(part 1 of 2)
# Autodesk Inventor assembly: Drive Roller Assembly 2
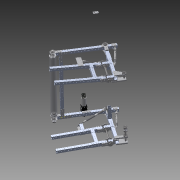
[picture p0: Inventor's stored thumbnail of the model, 180x180]
Saved by Autodesk Inventor 2014 (Build 180170000, 170)
## iProperties
Created: 2014-01-12
Part Number: Drive Roller Assembly 2
Document SubType Name: Assembly
Designer: Michael
Mass: 6489.5 g
Surface Area: 18387.5 cm^2
Volume: 1765.28 cm^3
Density: 3.67619 g/cm^3
Author: Michael
## Documents named in this file (45)
- C:\Users\Michael\Documents\GitHub\2014buildCAD\New Collector\Drive Roller Assembly 2.iam
- C:\Users\Michael\Documents\GitHub\2014buildCAD\Collector\Hex Shaft Collar 1-2 in (7552K500).ipt
- C:\Users\Michael\Documents\GitHub\2014buildCAD\Collector\Roller End Cap Drive (3-D Printed).ipt
- C:\Users\Michael\Documents\GitHub\2014buildCAD\Collector\VersaPlanetary (Fixed).iam
- C:\Users\Michael\Documents\GitHub\2014buildCAD\New Collector\Polycarbonate Roller 2 OD 1-16 Thick (8585K64).ipt
- C:\Users\Michael\Documents\GitHub\2014buildCAD\New Collector\Hex Bearing 1-2 in (FR8ZZ-Hex, am-0279).ipt
- C:\Users\Michael\Documents\GitHub\2014buildCAD\New Collector\Hex Shaft Collar 1-2 in (7552K500).ipt
- C:\Users\Michael\Documents\GitHub\2014buildCAD\New Collector\Roller End Cap Drive (3-D Printed).ipt
- C:\Users\Michael\Documents\GitHub\2014buildCAD\New Collector\Vex Pro End Bearing Mount.ipt
- C:\Users\Michael\Documents\GitHub\2014buildCAD\New Collector\Vex Pro 1x1 rectangular tubing 14 in length.ipt
- C:\Users\Michael\Documents\GitHub\2014buildCAD\New Collector\Hex Shaft Aluminum 1-2 in (am-2291).ipt
- C:\Users\Michael\Documents\GitHub\2014buildCAD\New Collector\Timing Pulley (HTD 5mm) - 18T 9mm Double Flange, 1-2 in Hex (VexPro).ipt
- C:\Users\Michael\Documents\GitHub\2014buildCAD\New Collector\Clamp with Piston Assembly.iam
- C:\Users\Michael\Documents\GitHub\2014buildCAD\New Collector\Vex Pro 90 degree gusset.ipt
- C:\Users\Michael\Documents\GitHub\2014buildCAD\New Collector\Vex Pro 1x1 rectangular tubing 2 in length.ipt
- C:\Users\Michael\Documents\GitHub\2014buildCAD\New Collector\Hex Shaft 3-8 in (am-0855).ipt
- C:\Users\Michael\Documents\GitHub\2014buildCAD\New Collector\Hex Shaft Collar 3-8 in (7552K300).ipt
- C:\Users\Michael\Documents\GitHub\2014buildCAD\New Collector\Hex Shaft 1-2 in (am-0856).ipt
- C:\Users\Michael\Documents\GitHub\2014buildCAD\New Collector\Spacer 2.ipt
- C:\Users\Michael\Documents\GitHub\2014buildCAD\New Collector\Gusset 3 (R-R) (Custom) ipt.ipt
- C:\Users\Michael\Documents\GitHub\2014buildCAD\New Collector\Gusset 3 (L-R) (Custom).ipt
- C:\Users\Michael\Documents\GitHub\2014buildCAD\New Collector\Gusset 3 (L-L) (Custom) ipt.ipt
- C:\Users\Michael\Documents\GitHub\2014buildCAD\New Collector\Gusset 3 (R-L) (Custom).ipt
- C:\Users\Michael\Documents\GitHub\2014buildCAD\New Collector\Vex Pro 1x1 rectangular tubing 4 in length.ipt
- C:\Users\Michael\Documents\GitHub\2014buildCAD\New Collector\Pneumatic Piston Front Flange (Lt Custom).ipt
- C:\Users\Michael\Documents\GitHub\2014buildCAD\New Collector\Pneumatic Piston Front Flange (Rt Custom).ipt
- C:\Users\Michael\Documents\GitHub\2014buildCAD\New Collector\Pneumatic Piston Back Flange (Rt Custom).ipt
- C:\Users\Michael\Documents\GitHub\2014buildCAD\New Collector\Bearing Mount Spacer 1-8 in.ipt
- C:\Users\Michael\Documents\GitHub\2014buildCAD\New Collector\Vex Pro 1x1 rectangular tubing 14 in length (roller).ipt
- C:\Users\Michael\Documents\GitHub\2014buildCAD\New Collector\Pneumatic Piston Back Flange (Right Custom).ipt
- C:\Users\Michael\Documents\GitHub\2014buildCAD\New Collector\Hex Shaft 1-2 in 5 in long (am-0856).ipt
- C:\Users\Michael\Documents\GitHub\2014buildCAD\New Collector\Vex Pro End Bearing Mount (Bolt).ipt
- C:\Users\Michael\Documents\GitHub\2014buildCAD\New Collector\Bracket.ipt
- C:\Users\Michael\Documents\GitHub\2014buildCAD\New Collector\Roller Piston 4 (.5 and 1 in Stroke, 9-16 in Bore).iam
- C:\Users\Michael\Documents\GitHub\2014buildCAD\New Collector\Shaft Collar 3-16 in ID (6435K510).ipt
- C:\Users\Michael\Documents\GitHub\2014buildCAD\New Collector\Standoff #8 (91125A459).ipt
- C:\Users\Michael\Documents\GitHub\2014buildCAD\New Collector\Vex Pro 1x1 rectangular tubing 21.375 in length.ipt
- C:\Users\Michael\Documents\GitHub\2014buildCAD\New Collector\Roller Crossbar Gusset (Custom).ipt
- C:\Users\Michael\Documents\GitHub\2014buildCAD\New Collector\Vex Pro 1x1 rectangular tubing 2 in length (Flange Support).ipt
- C:\Users\Michael\Documents\GitHub\2014buildCAD\New Collector\Vex Pro 90 degree gusset (1-8 in).ipt
- C:\Users\Michael\Documents\GitHub\2014buildCAD\New Collector\Timing Pulley (HTD 5mm) - 18T 15mm 1-2 in Hex.ipt
- C:\Users\Michael\Documents\GitHub\2014buildCAD\New Collector\Hex Spacer.ipt
- C:\Users\Michael\Documents\GitHub\2014buildCAD\New Collector\Side Mount Custom.ipt
- C:\Users\Michael\Documents\GitHub\2014buildCAD\New Collector\Clamp Piston ( 1 in stroke twice, 9-16 bore).iam
- C:\Users\Michael\Documents\GitHub\2014buildCAD\New Collector\Hex Spacer 1-2 .ipt
## Components (138 placed, 42 different names)
1. Roller End Cap Drive (3-D Printed):2 — Mate:154, Mate:155, Mate:157, Mate:158, Mate:466, Mate:469
2. VersaPlanetary (Fixed):1 [sub-assembly] — Mate:113, Mate:114, Mate:120, Mate:121, Mate:153, Mate:990, Mate:991, Mate:992
3. Hex Shaft Collar 1-2 in (7552K500):9 — Mate:113, Mate:114
4. Hex Shaft Collar 1-2 in (7552K500):10 — Mate:120, Mate:121
5. Polycarbonate Roller 2 OD 1-16 Thick (8585K64):3 — Mate:157, Mate:158, Mate:159, Mate:160
6. Hex Bearing 1-2 in (FR8ZZ-Hex, am-0279):3 — Mate:128, Mate:129, Mate:134, Mate:466, Mate:797
7. Roller End Cap Drive (3-D Printed):5 — Mate:159, Mate:160, Mate:632, Mate:635
8. Hex Shaft Aluminum 1-2 in (am-2291):1 — Flush:1, Mate:132, Mate:133, Mate:134, Mate:143, Mate:144, Mate:146, Mate:147, Mate:154, Mate:155, Mate:172, Mate:173, Mate:179, Mate:180, Mate:467, Mate:468, Mate:797
9. Vex Pro End Bearing Mount:4 — Mate:130, Mate:131, Mate:621, Mate:798, Mate:799, Mate:873
10. Vex Pro End Bearing Mount:5 — Mate:128, Mate:129, Mate:624, Mate:800, Mate:801, Mate:866, Mate:867, Mate:868, Mate:869, Mate:870, Mate:871, Mate:872
11. Hex Bearing 1-2 in (FR8ZZ-Hex, am-0279):4 — Mate:130, Mate:131, Flush:1, Mate:132, Mate:133, Mate:161
12. Timing Pulley (HTD 5mm) - 18T 9mm Double Flange, 1-2 in Hex (VexPro):3 — Mate:143, Mate:144, Mate:145, Mate:161
13. Hex Shaft Collar 1-2 in (7552K500):13 — Mate:145, Mate:146, Mate:147, Flush:2
14. Hex Shaft Collar 1-2 in (7552K500):14 — Flush:4, Mate:152
15. Timing Pulley (HTD 5mm) - 18T 9mm Double Flange, 1-2 in Hex (VexPro):4 — Mate:150, Flush:3, Mate:151, Flush:4, Mate:152
16. Hex Shaft Collar 1-2 in (7552K500):15 — Flush:2, Mate:150, Flush:3, Mate:151, Mate:153
17. Hex Bearing 1-2 in (FR8ZZ-Hex, am-0279):5 — Mate:178, Mate:758, Mate:759
18. Vex Pro End Bearing Mount:7 — Mate:631, Mate:804, Mate:805
19. Vex Pro End Bearing Mount:8 — Mate:629, Mate:802, Mate:803, Mate:874, Mate:875, Mate:876, Mate:877, Mate:878, Mate:879, Mate:880, Mate:881
20. Hex Bearing 1-2 in (FR8ZZ-Hex, am-0279):6 — Mate:172, Mate:173, Mate:470, Mate:471, Mate:632
21. Hex Shaft Collar 1-2 in (7552K500):16 — Mate:178, Mate:179, Mate:180, Flush:13
22. Clamp with Piston Assembly:1 [sub-assembly] — Mate:226, Mate:227, Flush:6, Mate:230, Mate:233, Mate:673, Mate:689, Mate:690, Mate:918, Mate:921
23. Vex Pro 1x1 rectangular tubing 14 in length:5 — Mate:203, Mate:210, Mate:211, Mate:221, Mate:222, Mate:223, Mate:427, Mate:429, Flush:20, Mate:653, Mate:940, Mate:942, Mate:975, Mate:979, Mate:981, Mate:983, Mate:1022, Mate:1023, Flush:27, Mate:1053, Mate:1054, Mate:1055
24. Vex Pro 1x1 rectangular tubing 14 in length:6 — Mate:258, Mate:259, Mate:260, Mate:263, Mate:320, Mate:321, Mate:418, Mate:419, Mate:420, Flush:20, Mate:658, Mate:935, Mate:936, Mate:938, Mate:973, Mate:974, Mate:976, Mate:977, Mate:978, Mate:1020, Mate:1021, Flush:26, Mate:1056, Mate:1057, Mate:1058
25. Vex Pro 90 degree gusset:8 — Mate:203, Mate:210, Mate:211, Mate:212, Mate:213, Mate:214
26. Vex Pro 1x1 rectangular tubing 2 in length:1 — Mate:212, Mate:213, Mate:214, Flush:25, Mate:941, Mate:961, Mate:962, Mate:964, Mate:965
27. Vex Pro 90 degree gusset:10 — Mate:221, Mate:222, Mate:223, Mate:433, Mate:434, Mate:435
28. Vex Pro 1x1 rectangular tubing 2 in length:2 — Mate:224, Mate:225, Flush:5, Mate:428, Mate:967, Mate:968, Mate:970, Mate:971
29. Hex Shaft 3-8 in (am-0855):1 — Mate:224, Mate:225, Flush:5, Mate:226, Mate:227, Flush:6, Mate:228, Mate:229, Mate:231, Mate:232, Mate:919, Mate:920, Mate:922, Mate:923, Mate:963, Mate:966, Mate:969, Mate:972
30. Hex Shaft Collar 3-8 in (7552K300):1 — Mate:228, Mate:229, Mate:230
31. Hex Shaft Collar 3-8 in (7552K300):2 — Mate:231, Mate:232, Mate:233
32. Clamp with Piston Assembly:2 [sub-assembly] — Mate:666, Mate:668, Mate:669, Mate:916, Mate:924
33. Vex Pro 90 degree gusset:12 — Mate:263, Mate:320, Mate:321, Mate:324, Mate:325
34. Vex Pro 1x1 rectangular tubing 2 in length:3 — Mate:324, Mate:325, Flush:25, Mate:937, Mate:949, Mate:950, Mate:952, Mate:953
35. Vex Pro 90 degree gusset:13 — Mate:258, Mate:259, Mate:260, Mate:425, Mate:426, Mate:492
36. Vex Pro 1x1 rectangular tubing 2 in length:4 — Mate:955, Mate:956, Mate:958, Mate:959
37. Hex Shaft 3-8 in (am-0855):2 — Mate:915, Mate:917, Mate:925, Mate:926, Mate:951, Mate:954, Mate:957, Mate:960
38. Hex Shaft Collar 3-8 in (7552K300):3
39. Hex Shaft Collar 3-8 in (7552K300):4
40. Vex Pro 90 degree gusset:14 — Mate:476, Mate:477, Mate:478, Mate:653
41. Vex Pro 90 degree gusset:15 — Mate:650, Mate:651, Mate:652, Mate:939, Mate:1022, Mate:1023
42. Vex Pro 90 degree gusset:17 — Mate:485, Mate:486, Mate:487
43. Vex Pro 90 degree gusset:18 — Mate:656, Mate:657, Mate:658, Mate:659, Mate:1020, Mate:1021
44. Hex Shaft 1-2 in (am-0856):2 — Mate:402, Mate:403, Mate:405, Mate:406, Mate:447, Mate:448, Flush:12
45. Hex Shaft Collar 1-2 in (7552K500):18 — Mate:402, Mate:403, Mate:450, Flush:12
46. Hex Shaft Collar 1-2 in (7552K500):19 — Mate:405, Mate:406, Mate:449
47. Hex Shaft Collar 1-2 in (7552K500):20 — Mate:706, Mate:707, Mate:726, Mate:945
48. Hex Shaft Collar 1-2 in (7552K500):21 — Mate:446, Mate:704, Mate:705, Flush:22
49. Spacer 2:1 — Mate:418, Mate:419, Mate:420, Mate:438, Mate:439, Mate:451, Mate:452, Mate:453
50. Gusset 3 (R-R) (Custom) ipt:1 — Mate:425, Mate:426, Mate:446, Mate:492
51. Spacer 2:2 — Mate:427, Mate:428, Mate:429, Mate:430, Mate:431, Mate:455, Mate:456, Mate:457
52. Gusset 3 (L-R) (Custom):1 — Mate:430, Mate:431, Mate:447, Mate:448, Mate:450, Mate:461
53. Gusset 3 (L-L) (Custom) ipt:1 — Mate:433, Mate:434, Mate:435, Mate:449
54. Gusset 3 (R-L) (Custom):1 — Mate:438, Mate:439, Mate:465, Mate:708, Mate:709, Mate:726, Mate:1034
55. Spacer 2:3 — Mate:451, Mate:452, Mate:453, Mate:462, Mate:463, Mate:464
56. Spacer 2:4 — Mate:455, Mate:456, Mate:457, Mate:458, Mate:459, Mate:460
57. Spacer 2:5 — Mate:458, Mate:459, Mate:460, Mate:461
58. Spacer 2:6 — Mate:462, Mate:463, Mate:464, Mate:465
59. Hex Shaft Collar 1-2 in (7552K500):22 — Mate:467, Mate:468, Mate:469
60. Hex Shaft Aluminum 1-2 in (am-2291):2 — Mate:470, Mate:471, Flush:13, Mate:633, Mate:634, Mate:758, Mate:759
61. Vex Pro 1x1 rectangular tubing 4 in length:1 — Mate:476, Mate:477, Mate:478, Mate:650, Mate:651, Mate:652, Mate:683, Mate:684, Mate:685
62. Vex Pro 1x1 rectangular tubing 4 in length:2 — Mate:485, Mate:486, Mate:487, Mate:656, Mate:657, Mate:659, Mate:694, Mate:699, Mate:700
63. Bearing Mount Spacer 1-8 in:1 — Mate:748, Mate:749, Mate:750, Mate:973, Mate:976
64. Bearing Mount Spacer 1-8 in:3 — Mate:743, Mate:744, Mate:745, Mate:974, Mate:978
65. Hex Bearing 1-2 in (FR8ZZ-Hex, am-0279):7 — Flush:15, Mate:560, Mate:561, Flush:23, Mate:754, Mate:755, Mate:830
66. Hex Shaft 1-2 in (am-0856):4 — Mate:560, Mate:561, Mate:562, Mate:563, Flush:23, Mate:774, Mate:829, Mate:831, Mate:833, Mate:834, Mate:1040, Mate:1043
67. Hex Bearing 1-2 in (FR8ZZ-Hex, am-0279):8 — Flush:15, Mate:746, Mate:747, Mate:774, Mate:832
68. Vex Pro 1x1 rectangular tubing 14 in length (roller):1 — Mate:562, Mate:563, Mate:621, Mate:624, Flush:21, Mate:790, Mate:791, Mate:793, Mate:798, Mate:799, Mate:800, Mate:801, Mate:862, Mate:863, Mate:864, Mate:887, Mate:903, Mate:904, Mate:909, Mate:910, Mate:912, Mate:988, Mate:989, Mate:1038, Mate:1039, Mate:1041, Mate:1042, Flush:26, Mate:1050
69. Bearing Mount Spacer 1-8 in:5 — Mate:740, Mate:741, Mate:742, Mate:983
70. Bearing Mount Spacer 1-8 in:7 — Mate:735, Mate:736, Mate:737, Mate:975, Mate:980
71. Hex Bearing 1-2 in (FR8ZZ-Hex, am-0279):9 — Flush:19, Mate:752, Mate:753, Mate:854
72. Hex Shaft 1-2 in (am-0856):5 — Flush:19, Mate:775, Mate:836, Mate:843, Mate:852, Mate:853, Mate:1037, Mate:1046, Mate:1049
73. Hex Bearing 1-2 in (FR8ZZ-Hex, am-0279):10 — Mate:738, Mate:739, Mate:775, Mate:835
74. Vex Pro 1x1 rectangular tubing 14 in length (roller):2 — Mate:629, Mate:631, Flush:21, Mate:802, Mate:803, Mate:804, Mate:805, Mate:806, Mate:807, Mate:808, Mate:809, Mate:810, Mate:811, Mate:892, Mate:896, Mate:905, Mate:906, Mate:907, Mate:908, Mate:1036, Mate:1044, Mate:1045, Mate:1047, Mate:1048, Flush:27
75. Hex Shaft Collar 1-2 in (7552K500):23 — Mate:633, Mate:634, Mate:635
76. Pneumatic Piston Front Flange (Rt Custom):2 — Mate:666, Mate:668, Mate:669, Mate:932, Mate:933, Mate:934, Mate:1051
77. Pneumatic Piston Front Flange (Lt Custom):1 — Mate:673, Mate:689, Mate:690, Mate:929, Mate:930, Mate:931, Mate:1052
78. Pneumatic Piston Back Flange (Rt Custom):1 — Mate:683, Mate:684, Mate:685, Mate:1028, Mate:1029, Mate:1030
79. Pneumatic Piston Back Flange (Right Custom):1 — Mate:694, Mate:699, Mate:700, Mate:1024, Mate:1025, Mate:1026
80. Hex Shaft 1-2 in 5 in long (am-0856):1 — Mate:704, Mate:705, Mate:706, Mate:707, Mate:708, Mate:709, Flush:22, Mate:714, Mate:715, Mate:946, Mate:947, Mate:1032, Mate:1033
81. Hex Shaft Collar 1-2 in (7552K500):24 — Mate:714, Mate:715, Mate:948
82. Vex Pro End Bearing Mount (Bolt):1 — Mate:735, Mate:736, Mate:737, Mate:738, Mate:739, Mate:979, Mate:980
83. Vex Pro End Bearing Mount (Bolt):2 — Mate:740, Mate:741, Mate:742, Mate:752, Mate:753, Mate:981
84. Vex Pro End Bearing Mount (Bolt):3 — Mate:743, Mate:744, Mate:745, Mate:746, Mate:747
85. Vex Pro End Bearing Mount (Bolt):4 — Mate:748, Mate:749, Mate:750, Mate:754, Mate:755, Mate:977
86. Bracket:1 — Mate:790, Mate:791, Mate:793, Mate:860, Mate:1059
87. Bracket:2 — Mate:806, Mate:807, Mate:808, Mate:856, Mate:1060
88. Bracket:3 — Mate:809, Mate:810, Mate:811, Mate:858
89. Hex Shaft Collar 1-2 in (7552K500):25 — Mate:829, Mate:830, Mate:831
90. Hex Shaft Collar 1-2 in (7552K500):26 — Mate:832, Mate:833, Mate:834
91. Hex Shaft Collar 1-2 in (7552K500):27 — Mate:835, Mate:836, Mate:843
92. Hex Shaft Collar 1-2 in (7552K500):29 — Mate:852, Mate:853, Mate:854
93. Shaft Collar 3-16 in ID (6435K510):1 — Mate:858, Mate:1062
94. Shaft Collar 3-16 in ID (6435K510):2 — Mate:856, Mate:1061
95. Shaft Collar 3-16 in ID (6435K510):3 — Mate:860, Mate:1063
96. Shaft Collar 3-16 in ID (6435K510):4 — Mate:865, Mate:1064
97. Bracket:4 — Mate:862, Mate:863, Mate:864, Mate:865
98. Standoff #8 (91125A459):1 — Mate:866, Mate:867
99. Standoff #8 (91125A459):2 — Mate:868, Mate:869
100. Standoff #8 (91125A459):3 — Mate:870, Mate:871
101. Standoff #8 (91125A459):4 — Mate:872, Mate:873
102. Standoff #8 (91125A459):5 — Mate:874, Mate:875
103. Standoff #8 (91125A459):6 — Mate:876, Mate:877
104. Standoff #8 (91125A459):7 — Mate:878, Mate:879
105. Standoff #8 (91125A459):8 — Mate:880, Mate:881
106. Vex Pro 1x1 rectangular tubing 21.375 in length:1 — Mate:894, Mate:897, Mate:900, Mate:901, Mate:902, Mate:911
107. Roller Crossbar Gusset (Custom):2 — Mate:887, Mate:900, Mate:901, Mate:902, Mate:903, Mate:904
108. Roller Crossbar Gusset (Custom):3 — Mate:896, Mate:897, Mate:905, Mate:906
109. Roller Crossbar Gusset (Custom):4 — Mate:892, Mate:894, Mate:907, Mate:908
110. Roller Crossbar Gusset (Custom):5 — Mate:909, Mate:910, Mate:911, Mate:912
111. Hex Shaft Collar 3-8 in (7552K300):5 — Mate:915, Mate:916, Mate:917
112. Hex Shaft Collar 3-8 in (7552K300):6 — Mate:918, Mate:919, Mate:920
113. Hex Shaft Collar 3-8 in (7552K300):7 — Mate:921, Mate:922, Mate:923
114. Hex Shaft Collar 3-8 in (7552K300):8 — Mate:924, Mate:925, Mate:926
115. Vex Pro 1x1 rectangular tubing 2 in length (Flange Support):1 — Mate:929, Mate:930, Mate:931
116. Vex Pro 1x1 rectangular tubing 2 in length (Flange Support):2 — Mate:932, Mate:933, Mate:934
117. Vex Pro 90 degree gusset (1-8 in):1 — Mate:935, Mate:936, Mate:937, Mate:938
118. Vex Pro 90 degree gusset (1-8 in):2 — Mate:939, Mate:940, Mate:941, Mate:942
119. Timing Pulley (HTD 5mm) - 18T 15mm 1-2 in Hex:1 — Mate:945, Mate:946, Mate:947, Mate:948
120. Hex Spacer:1 — Mate:949, Mate:950, Mate:951
121. Hex Spacer:2 — Mate:952, Mate:953, Mate:954
122. Hex Spacer:3 — Mate:955, Mate:956, Mate:957
123. Hex Spacer:4 — Mate:958, Mate:959, Mate:960
124. Hex Spacer:5 — Mate:961, Mate:962, Mate:963
125. Hex Spacer:6 — Mate:964, Mate:965, Mate:966
126. Hex Spacer:7 — Mate:967, Mate:968, Mate:969
127. Hex Spacer:8 — Mate:970, Mate:971, Mate:972
128. Side Mount Custom:1 — Mate:988, Mate:989, Mate:990, Mate:991, Mate:992, Mate:1050
129. Clamp Piston ( 1 in stroke twice, 9-16 bore):1 [sub-assembly] — Mate:1024, Mate:1025, Mate:1026, Mate:1051
130. Clamp Piston ( 1 in stroke twice, 9-16 bore):2 [sub-assembly] — Mate:1028, Mate:1029, Mate:1030, Mate:1052
131. Hex Shaft Collar 1-2 in (7552K500):30 — Mate:1032, Mate:1033, Mate:1034
132. Hex Spacer:9 — Mate:1036, Mate:1037
133. Hex Spacer 1-2 :1 — Mate:1038, Mate:1039, Mate:1040
134. Hex Spacer 1-2 :2 — Mate:1041, Mate:1042, Mate:1043
135. Hex Spacer 1-2 :3 — Mate:1044, Mate:1045, Mate:1046
136. Hex Spacer 1-2 :4 — Mate:1047, Mate:1048, Mate:1049
137. Roller Piston 4 (.5 and 1 in Stroke, 9-16 in Bore):1 [sub-assembly] — Mate:1053, Mate:1054, Mate:1055, Mate:1060, Mate:1061, Mate:1062
138. Roller Piston 4 (.5 and 1 in Stroke, 9-16 in Bore):2 [sub-assembly] — Mate:1056, Mate:1057, Mate:1058, Mate:1059, Mate:1063, Mate:1064
## Relationships (404: Mate 384, Flush 20)
- Mate:113: VersaPlanetary (Fixed):1 ↔ Hex Shaft Collar 1-2 in (7552K500):9
- Mate:114: VersaPlanetary (Fixed):1 ↔ Hex Shaft Collar 1-2 in (7552K500):9
- Mate:120: VersaPlanetary (Fixed):1 ↔ Hex Shaft Collar 1-2 in (7552K500):10
- Mate:121: VersaPlanetary (Fixed):1 ↔ Hex Shaft Collar 1-2 in (7552K500):10
- Mate:128: Hex Bearing 1-2 in (FR8ZZ-Hex, am-0279):3 ↔ Vex Pro End Bearing Mount:5
- Mate:129: Hex Bearing 1-2 in (FR8ZZ-Hex, am-0279):3 ↔ Vex Pro End Bearing Mount:5
- Mate:130: Vex Pro End Bearing Mount:4 ↔ Hex Bearing 1-2 in (FR8ZZ-Hex, am-0279):4
- Mate:131: Vex Pro End Bearing Mount:4 ↔ Hex Bearing 1-2 in (FR8ZZ-Hex, am-0279):4
- Flush:1 (-25.4 mm): Hex Shaft Aluminum 1-2 in (am-2291):1 ↔ Hex Bearing 1-2 in (FR8ZZ-Hex, am-0279):4
- Mate:132: Hex Shaft Aluminum 1-2 in (am-2291):1 ↔ Hex Bearing 1-2 in (FR8ZZ-Hex, am-0279):4
- Mate:133: Hex Shaft Aluminum 1-2 in (am-2291):1 ↔ Hex Bearing 1-2 in (FR8ZZ-Hex, am-0279):4
- Mate:134: Hex Bearing 1-2 in (FR8ZZ-Hex, am-0279):3 ↔ Hex Shaft Aluminum 1-2 in (am-2291):1
- Mate:143: Hex Shaft Aluminum 1-2 in (am-2291):1 ↔ Timing Pulley (HTD 5mm) - 18T 9mm Double Flange, 1-2 in Hex (VexPro):3
- Mate:144: Hex Shaft Aluminum 1-2 in (am-2291):1 ↔ Timing Pulley (HTD 5mm) - 18T 9mm Double Flange, 1-2 in Hex (VexPro):3
- Mate:145: Timing Pulley (HTD 5mm) - 18T 9mm Double Flange, 1-2 in Hex (VexPro):3 ↔ Hex Shaft Collar 1-2 in (7552K500):13
- Mate:146: Hex Shaft Aluminum 1-2 in (am-2291):1 ↔ Hex Shaft Collar 1-2 in (7552K500):13
- Mate:147: Hex Shaft Aluminum 1-2 in (am-2291):1 ↔ Hex Shaft Collar 1-2 in (7552K500):13
- [Mate]: Hex Shaft Collar 1-2 in (7552K500):14 ↔ Timing Pulley (HTD 5mm) - 18T 9mm Double Flange, 1-2 in Hex (VexPro):4
- [Mate]: Timing Pulley (HTD 5mm) - 18T 9mm Double Flange, 1-2 in Hex (VexPro):4 ↔ Hex Shaft Collar 1-2 in (7552K500):15
- Flush:2: Hex Shaft Collar 1-2 in (7552K500):13 ↔ Hex Shaft Collar 1-2 in (7552K500):15
- Mate:150: Timing Pulley (HTD 5mm) - 18T 9mm Double Flange, 1-2 in Hex (VexPro):4 ↔ Hex Shaft Collar 1-2 in (7552K500):15
- Flush:3: Timing Pulley (HTD 5mm) - 18T 9mm Double Flange, 1-2 in Hex (VexPro):4 ↔ Hex Shaft Collar 1-2 in (7552K500):15
- Mate:151: Timing Pulley (HTD 5mm) - 18T 9mm Double Flange, 1-2 in Hex (VexPro):4 ↔ Hex Shaft Collar 1-2 in (7552K500):15
- Flush:4: Hex Shaft Collar 1-2 in (7552K500):14 ↔ Timing Pulley (HTD 5mm) - 18T 9mm Double Flange, 1-2 in Hex (VexPro):4
- Mate:152: Hex Shaft Collar 1-2 in (7552K500):14 ↔ Timing Pulley (HTD 5mm) - 18T 9mm Double Flange, 1-2 in Hex (VexPro):4
- Mate:153: VersaPlanetary (Fixed):1 ↔ Hex Shaft Collar 1-2 in (7552K500):15
- Mate:154: Roller End Cap Drive (3-D Printed):2 ↔ Hex Shaft Aluminum 1-2 in (am-2291):1
- Mate:155: Roller End Cap Drive (3-D Printed):2 ↔ Hex Shaft Aluminum 1-2 in (am-2291):1
- Mate:157: Roller End Cap Drive (3-D Printed):2 ↔ Polycarbonate Roller 2 OD 1-16 Thick (8585K64):3
- Mate:158: Roller End Cap Drive (3-D Printed):2 ↔ Polycarbonate Roller 2 OD 1-16 Thick (8585K64):3
- Mate:159: Polycarbonate Roller 2 OD 1-16 Thick (8585K64):3 ↔ Roller End Cap Drive (3-D Printed):5
- Mate:160: Polycarbonate Roller 2 OD 1-16 Thick (8585K64):3 ↔ Roller End Cap Drive (3-D Printed):5
- Mate:161: Hex Bearing 1-2 in (FR8ZZ-Hex, am-0279):4 ↔ Timing Pulley (HTD 5mm) - 18T 9mm Double Flange, 1-2 in Hex (VexPro):3
- [Mate]: Hex Bearing 1-2 in (FR8ZZ-Hex, am-0279):5 ↔ Vex Pro End Bearing Mount:8
- [Mate]: Hex Bearing 1-2 in (FR8ZZ-Hex, am-0279):5 ↔ Vex Pro End Bearing Mount:8
- [Mate]: Vex Pro End Bearing Mount:7 ↔ Hex Bearing 1-2 in (FR8ZZ-Hex, am-0279):6
- [Mate]: Vex Pro End Bearing Mount:7 ↔ Hex Bearing 1-2 in (FR8ZZ-Hex, am-0279):6
- Mate:172: Hex Shaft Aluminum 1-2 in (am-2291):1 ↔ Hex Bearing 1-2 in (FR8ZZ-Hex, am-0279):6
- Mate:173: Hex Shaft Aluminum 1-2 in (am-2291):1 ↔ Hex Bearing 1-2 in (FR8ZZ-Hex, am-0279):6
- Mate:178: Hex Bearing 1-2 in (FR8ZZ-Hex, am-0279):5 ↔ Hex Shaft Collar 1-2 in (7552K500):16
- Mate:179: Hex Shaft Aluminum 1-2 in (am-2291):1 ↔ Hex Shaft Collar 1-2 in (7552K500):16
- Mate:180: Hex Shaft Aluminum 1-2 in (am-2291):1 ↔ Hex Shaft Collar 1-2 in (7552K500):16
- Mate:203: Vex Pro 1x1 rectangular tubing 14 in length:5 ↔ Vex Pro 90 degree gusset:8
- Mate:210: Vex Pro 1x1 rectangular tubing 14 in length:5 ↔ Vex Pro 90 degree gusset:8
- Mate:211: Vex Pro 1x1 rectangular tubing 14 in length:5 ↔ Vex Pro 90 degree gusset:8
- Mate:212: Vex Pro 90 degree gusset:8 ↔ Vex Pro 1x1 rectangular tubing 2 in length:1
- Mate:213: Vex Pro 90 degree gusset:8 ↔ Vex Pro 1x1 rectangular tubing 2 in length:1
- Mate:214: Vex Pro 90 degree gusset:8 ↔ Vex Pro 1x1 rectangular tubing 2 in length:1
- [Mate]: Vex Pro 90 degree gusset:10 ↔ Vex Pro 1x1 rectangular tubing 2 in length:2
- [Mate]: Vex Pro 90 degree gusset:10 ↔ Vex Pro 1x1 rectangular tubing 2 in length:2
- [Mate]: Vex Pro 90 degree gusset:10 ↔ Vex Pro 1x1 rectangular tubing 2 in length:2
- Mate:221: Vex Pro 1x1 rectangular tubing 14 in length:5 ↔ Vex Pro 90 degree gusset:10
- Mate:222: Vex Pro 1x1 rectangular tubing 14 in length:5 ↔ Vex Pro 90 degree gusset:10
- Mate:223: Vex Pro 1x1 rectangular tubing 14 in length:5 ↔ Vex Pro 90 degree gusset:10
- Mate:224: Vex Pro 1x1 rectangular tubing 2 in length:2 ↔ Hex Shaft 3-8 in (am-0855):1
- Mate:225: Vex Pro 1x1 rectangular tubing 2 in length:2 ↔ Hex Shaft 3-8 in (am-0855):1
- Flush:5 (-19.05 mm): Vex Pro 1x1 rectangular tubing 2 in length:2 ↔ Hex Shaft 3-8 in (am-0855):1
- Mate:226: Clamp with Piston Assembly:1 ↔ Hex Shaft 3-8 in (am-0855):1
- Mate:227: Clamp with Piston Assembly:1 ↔ Hex Shaft 3-8 in (am-0855):1
- Flush:6 (-7.1437 mm): Clamp with Piston Assembly:1 ↔ Hex Shaft 3-8 in (am-0855):1
- Mate:228: Hex Shaft 3-8 in (am-0855):1 ↔ Hex Shaft Collar 3-8 in (7552K300):1
- Mate:229: Hex Shaft 3-8 in (am-0855):1 ↔ Hex Shaft Collar 3-8 in (7552K300):1
- Mate:230: Clamp with Piston Assembly:1 ↔ Hex Shaft Collar 3-8 in (7552K300):1
- Mate:231: Hex Shaft 3-8 in (am-0855):1 ↔ Hex Shaft Collar 3-8 in (7552K300):2
- Mate:232: Hex Shaft 3-8 in (am-0855):1 ↔ Hex Shaft Collar 3-8 in (7552K300):2
- Mate:233: Clamp with Piston Assembly:1 ↔ Hex Shaft Collar 3-8 in (7552K300):2
- [Mate]: Vex Pro 90 degree gusset:12 ↔ Vex Pro 1x1 rectangular tubing 2 in length:3
- [Mate]: Vex Pro 90 degree gusset:13 ↔ Vex Pro 1x1 rectangular tubing 2 in length:4
- [Mate]: Vex Pro 90 degree gusset:13 ↔ Vex Pro 1x1 rectangular tubing 2 in length:4
- [Mate]: Vex Pro 90 degree gusset:13 ↔ Vex Pro 1x1 rectangular tubing 2 in length:4
- [Mate]: Vex Pro 1x1 rectangular tubing 2 in length:4 ↔ Hex Shaft 3-8 in (am-0855):2
- [Mate]: Vex Pro 1x1 rectangular tubing 2 in length:4 ↔ Hex Shaft 3-8 in (am-0855):2
- [Flush] (-19.05 mm): Vex Pro 1x1 rectangular tubing 2 in length:4 ↔ Hex Shaft 3-8 in (am-0855):2
- [Mate]: Clamp with Piston Assembly:2 ↔ Hex Shaft 3-8 in (am-0855):2
- [Mate]: Clamp with Piston Assembly:2 ↔ Hex Shaft 3-8 in (am-0855):2
- [Flush] (-7.1437 mm): Clamp with Piston Assembly:2 ↔ Hex Shaft 3-8 in (am-0855):2
- [Mate]: Hex Shaft 3-8 in (am-0855):2 ↔ Hex Shaft Collar 3-8 in (7552K300):3
- [Mate]: Hex Shaft 3-8 in (am-0855):2 ↔ Hex Shaft Collar 3-8 in (7552K300):3
- [Mate]: Clamp with Piston Assembly:2 ↔ Hex Shaft Collar 3-8 in (7552K300):3
- [Mate]: Hex Shaft 3-8 in (am-0855):2 ↔ Hex Shaft Collar 3-8 in (7552K300):4
- [Mate]: Hex Shaft 3-8 in (am-0855):2 ↔ Hex Shaft Collar 3-8 in (7552K300):4
- [Mate]: Clamp with Piston Assembly:2 ↔ Hex Shaft Collar 3-8 in (7552K300):4
- Mate:258: Vex Pro 1x1 rectangular tubing 14 in length:6 ↔ Vex Pro 90 degree gusset:13
- Mate:259: Vex Pro 1x1 rectangular tubing 14 in length:6 ↔ Vex Pro 90 degree gusset:13
- Mate:260: Vex Pro 1x1 rectangular tubing 14 in length:6 ↔ Vex Pro 90 degree gusset:13
- Mate:263: Vex Pro 1x1 rectangular tubing 14 in length:6 ↔ Vex Pro 90 degree gusset:12
- Mate:320: Vex Pro 1x1 rectangular tubing 14 in length:6 ↔ Vex Pro 90 degree gusset:12
- Mate:321: Vex Pro 1x1 rectangular tubing 14 in length:6 ↔ Vex Pro 90 degree gusset:12
- Mate:324: Vex Pro 90 degree gusset:12 ↔ Vex Pro 1x1 rectangular tubing 2 in length:3
- Mate:325: Vex Pro 90 degree gusset:12 ↔ Vex Pro 1x1 rectangular tubing 2 in length:3
- Mate:402: Hex Shaft 1-2 in (am-0856):2 ↔ Hex Shaft Collar 1-2 in (7552K500):18
- Mate:403: Hex Shaft 1-2 in (am-0856):2 ↔ Hex Shaft Collar 1-2 in (7552K500):18
- Mate:405: Hex Shaft 1-2 in (am-0856):2 ↔ Hex Shaft Collar 1-2 in (7552K500):19
- Mate:406: Hex Shaft 1-2 in (am-0856):2 ↔ Hex Shaft Collar 1-2 in (7552K500):19
- Mate:418: Vex Pro 1x1 rectangular tubing 14 in length:6 ↔ Spacer 2:1
- Mate:419: Vex Pro 1x1 rectangular tubing 14 in length:6 ↔ Spacer 2:1
- Mate:420: Vex Pro 1x1 rectangular tubing 14 in length:6 ↔ Spacer 2:1
- Mate:425: Vex Pro 90 degree gusset:13 ↔ Gusset 3 (R-R) (Custom) ipt:1
- Mate:426: Vex Pro 90 degree gusset:13 ↔ Gusset 3 (R-R) (Custom) ipt:1
- Mate:427: Vex Pro 1x1 rectangular tubing 14 in length:5 ↔ Spacer 2:2
- Mate:428: Vex Pro 1x1 rectangular tubing 2 in length:2 ↔ Spacer 2:2
- Mate:429: Vex Pro 1x1 rectangular tubing 14 in length:5 ↔ Spacer 2:2
- Mate:430: Spacer 2:2 ↔ Gusset 3 (L-R) (Custom):1
- Mate:431: Spacer 2:2 ↔ Gusset 3 (L-R) (Custom):1
- Mate:433: Vex Pro 90 degree gusset:10 ↔ Gusset 3 (L-L) (Custom) ipt:1
- Mate:434: Vex Pro 90 degree gusset:10 ↔ Gusset 3 (L-L) (Custom) ipt:1
- Mate:435: Vex Pro 90 degree gusset:10 ↔ Gusset 3 (L-L) (Custom) ipt:1
- Mate:438: Spacer 2:1 ↔ Gusset 3 (R-L) (Custom):1
- Mate:439: Spacer 2:1 ↔ Gusset 3 (R-L) (Custom):1
- Mate:446: Hex Shaft Collar 1-2 in (7552K500):21 ↔ Gusset 3 (R-R) (Custom) ipt:1
- Mate:447: Hex Shaft 1-2 in (am-0856):2 ↔ Gusset 3 (L-R) (Custom):1
- Mate:448: Hex Shaft 1-2 in (am-0856):2 ↔ Gusset 3 (L-R) (Custom):1
- Mate:449: Hex Shaft Collar 1-2 in (7552K500):19 ↔ Gusset 3 (L-L) (Custom) ipt:1
- Mate:450: Hex Shaft Collar 1-2 in (7552K500):18 ↔ Gusset 3 (L-R) (Custom):1
- Mate:451: Spacer 2:1 ↔ Spacer 2:3
- Mate:452: Spacer 2:1 ↔ Spacer 2:3
- Mate:453: Spacer 2:1 ↔ Spacer 2:3
- Mate:455: Spacer 2:2 ↔ Spacer 2:4
- Mate:456: Spacer 2:2 ↔ Spacer 2:4
- Mate:457: Spacer 2:2 ↔ Spacer 2:4
- Mate:458: Spacer 2:4 ↔ Spacer 2:5
- Mate:459: Spacer 2:4 ↔ Spacer 2:5
- Mate:460: Spacer 2:4 ↔ Spacer 2:5
- Mate:461: Gusset 3 (L-R) (Custom):1 ↔ Spacer 2:5
- Mate:462: Spacer 2:3 ↔ Spacer 2:6
- Mate:463: Spacer 2:3 ↔ Spacer 2:6
- Mate:464: Spacer 2:3 ↔ Spacer 2:6
- Mate:465: Gusset 3 (R-L) (Custom):1 ↔ Spacer 2:6
- Flush:12 (-9.525 mm): Hex Shaft 1-2 in (am-0856):2 ↔ Hex Shaft Collar 1-2 in (7552K500):18
- Mate:466: Roller End Cap Drive (3-D Printed):2 ↔ Hex Bearing 1-2 in (FR8ZZ-Hex, am-0279):3
- Mate:467: Hex Shaft Aluminum 1-2 in (am-2291):1 ↔ Hex Shaft Collar 1-2 in (7552K500):22
- Mate:468: Hex Shaft Aluminum 1-2 in (am-2291):1 ↔ Hex Shaft Collar 1-2 in (7552K500):22
- Mate:469: Roller End Cap Drive (3-D Printed):2 ↔ Hex Shaft Collar 1-2 in (7552K500):22
- Mate:470: Hex Bearing 1-2 in (FR8ZZ-Hex, am-0279):6 ↔ Hex Shaft Aluminum 1-2 in (am-2291):2
- Mate:471: Hex Bearing 1-2 in (FR8ZZ-Hex, am-0279):6 ↔ Hex Shaft Aluminum 1-2 in (am-2291):2
- Flush:13 (-3.175 mm): Hex Shaft Collar 1-2 in (7552K500):16 ↔ Hex Shaft Aluminum 1-2 in (am-2291):2
- Mate:476: Vex Pro 90 degree gusset:14 ↔ Vex Pro 1x1 rectangular tubing 4 in length:1
- Mate:477: Vex Pro 90 degree gusset:14 ↔ Vex Pro 1x1 rectangular tubing 4 in length:1
- Mate:478: Vex Pro 90 degree gusset:14 ↔ Vex Pro 1x1 rectangular tubing 4 in length:1
- Mate:485: Vex Pro 90 degree gusset:17 ↔ Vex Pro 1x1 rectangular tubing 4 in length:2
- Mate:486: Vex Pro 90 degree gusset:17 ↔ Vex Pro 1x1 rectangular tubing 4 in length:2
- Mate:487: Vex Pro 90 degree gusset:17 ↔ Vex Pro 1x1 rectangular tubing 4 in length:2
- Mate:492: Vex Pro 90 degree gusset:13 ↔ Gusset 3 (R-R) (Custom) ipt:1
- Flush:15: Hex Bearing 1-2 in (FR8ZZ-Hex, am-0279):7 ↔ Hex Bearing 1-2 in (FR8ZZ-Hex, am-0279):8
- Mate:560: Hex Bearing 1-2 in (FR8ZZ-Hex, am-0279):7 ↔ Hex Shaft 1-2 in (am-0856):4
- Mate:561: Hex Bearing 1-2 in (FR8ZZ-Hex, am-0279):7 ↔ Hex Shaft 1-2 in (am-0856):4
- Mate:562: Hex Shaft 1-2 in (am-0856):4 ↔ Vex Pro 1x1 rectangular tubing 14 in length (roller):1
- Mate:563: Hex Shaft 1-2 in (am-0856):4 ↔ Vex Pro 1x1 rectangular tubing 14 in length (roller):1
- [Flush]: Hex Bearing 1-2 in (FR8ZZ-Hex, am-0279):9 ↔ Hex Bearing 1-2 in (FR8ZZ-Hex, am-0279):10
- [Mate]: Hex Bearing 1-2 in (FR8ZZ-Hex, am-0279):9 ↔ Hex Shaft 1-2 in (am-0856):5
- [Mate]: Hex Bearing 1-2 in (FR8ZZ-Hex, am-0279):9 ↔ Hex Shaft 1-2 in (am-0856):5
- [Mate]: Hex Shaft 1-2 in (am-0856):5 ↔ Vex Pro 1x1 rectangular tubing 14 in length (roller):2
- [Mate]: Hex Shaft 1-2 in (am-0856):5 ↔ Vex Pro 1x1 rectangular tubing 14 in length (roller):2
- Flush:19 (15.0812 mm): Hex Bearing 1-2 in (FR8ZZ-Hex, am-0279):9 ↔ Hex Shaft 1-2 in (am-0856):5
- Mate:621: Vex Pro End Bearing Mount:4 ↔ Vex Pro 1x1 rectangular tubing 14 in length (roller):1
- Mate:624: Vex Pro End Bearing Mount:5 ↔ Vex Pro 1x1 rectangular tubing 14 in length (roller):1
- Mate:629: Vex Pro End Bearing Mount:8 ↔ Vex Pro 1x1 rectangular tubing 14 in length (roller):2
- Flush:20: Vex Pro 1x1 rectangular tubing 14 in length:5 ↔ Vex Pro 1x1 rectangular tubing 14 in length:6
- Mate:631: Vex Pro End Bearing Mount:7 ↔ Vex Pro 1x1 rectangular tubing 14 in length (roller):2
- Mate:632: Roller End Cap Drive (3-D Printed):5 ↔ Hex Bearing 1-2 in (FR8ZZ-Hex, am-0279):6
- Mate:633: Hex Shaft Aluminum 1-2 in (am-2291):2 ↔ Hex Shaft Collar 1-2 in (7552K500):23
- Mate:634: Hex Shaft Aluminum 1-2 in (am-2291):2 ↔ Hex Shaft Collar 1-2 in (7552K500):23
- Mate:635: Roller End Cap Drive (3-D Printed):5 ↔ Hex Shaft Collar 1-2 in (7552K500):23
- Flush:21: Vex Pro 1x1 rectangular tubing 14 in length (roller):1 ↔ Vex Pro 1x1 rectangular tubing 14 in length (roller):2
- Mate:650: Vex Pro 90 degree gusset:15 ↔ Vex Pro 1x1 rectangular tubing 4 in length:1
- Mate:651: Vex Pro 90 degree gusset:15 ↔ Vex Pro 1x1 rectangular tubing 4 in length:1
- Mate:652: Vex Pro 90 degree gusset:15 ↔ Vex Pro 1x1 rectangular tubing 4 in length:1
- Mate:653: Vex Pro 1x1 rectangular tubing 14 in length:5 ↔ Vex Pro 90 degree gusset:14
- Mate:656: Vex Pro 90 degree gusset:18 ↔ Vex Pro 1x1 rectangular tubing 4 in length:2
- Mate:657: Vex Pro 90 degree gusset:18 ↔ Vex Pro 1x1 rectangular tubing 4 in length:2
- Mate:658: Vex Pro 1x1 rectangular tubing 14 in length:6 ↔ Vex Pro 90 degree gusset:18
- Mate:659: Vex Pro 90 degree gusset:18 ↔ Vex Pro 1x1 rectangular tubing 4 in length:2
- Mate:666: Clamp with Piston Assembly:2 ↔ Pneumatic Piston Front Flange (Rt Custom):2
- Mate:668: Clamp with Piston Assembly:2 ↔ Pneumatic Piston Front Flange (Rt Custom):2
- Mate:669: Clamp with Piston Assembly:2 ↔ Pneumatic Piston Front Flange (Rt Custom):2
- Mate:673: Clamp with Piston Assembly:1 ↔ Pneumatic Piston Front Flange (Lt Custom):1
- Mate:683: Vex Pro 1x1 rectangular tubing 4 in length:1 ↔ Pneumatic Piston Back Flange (Rt Custom):1
- Mate:684: Vex Pro 1x1 rectangular tubing 4 in length:1 ↔ Pneumatic Piston Back Flange (Rt Custom):1
- Mate:685: Vex Pro 1x1 rectangular tubing 4 in length:1 ↔ Pneumatic Piston Back Flange (Rt Custom):1
- Mate:689: Clamp with Piston Assembly:1 ↔ Pneumatic Piston Front Flange (Lt Custom):1
- Mate:690: Clamp with Piston Assembly:1 ↔ Pneumatic Piston Front Flange (Lt Custom):1
- Mate:694: Vex Pro 1x1 rectangular tubing 4 in length:2 ↔ Pneumatic Piston Back Flange (Right Custom):1
- Mate:699: Vex Pro 1x1 rectangular tubing 4 in length:2 ↔ Pneumatic Piston Back Flange (Right Custom):1
- Mate:700: Vex Pro 1x1 rectangular tubing 4 in length:2 ↔ Pneumatic Piston Back Flange (Right Custom):1
- Mate:704: Hex Shaft Collar 1-2 in (7552K500):21 ↔ Hex Shaft 1-2 in 5 in long (am-0856):1
- Mate:705: Hex Shaft Collar 1-2 in (7552K500):21 ↔ Hex Shaft 1-2 in 5 in long (am-0856):1
- Mate:706: Hex Shaft Collar 1-2 in (7552K500):20 ↔ Hex Shaft 1-2 in 5 in long (am-0856):1
- Mate:707: Hex Shaft Collar 1-2 in (7552K500):20 ↔ Hex Shaft 1-2 in 5 in long (am-0856):1
- Mate:708: Gusset 3 (R-L) (Custom):1 ↔ Hex Shaft 1-2 in 5 in long (am-0856):1
- Mate:709: Gusset 3 (R-L) (Custom):1 ↔ Hex Shaft 1-2 in 5 in long (am-0856):1
- Flush:22 (-3.175 mm): Hex Shaft Collar 1-2 in (7552K500):21 ↔ Hex Shaft 1-2 in 5 in long (am-0856):1
- Mate:714: Hex Shaft 1-2 in 5 in long (am-0856):1 ↔ Hex Shaft Collar 1-2 in (7552K500):24
- Mate:715: Hex Shaft 1-2 in 5 in long (am-0856):1 ↔ Hex Shaft Collar 1-2 in (7552K500):24
- Mate:726 (45.339 mm): Hex Shaft Collar 1-2 in (7552K500):20 ↔ Gusset 3 (R-L) (Custom):1
- Mate:735: Bearing Mount Spacer 1-8 in:7 ↔ Vex Pro End Bearing Mount (Bolt):1
- Mate:736: Bearing Mount Spacer 1-8 in:7 ↔ Vex Pro End Bearing Mount (Bolt):1
- Mate:737: Bearing Mount Spacer 1-8 in:7 ↔ Vex Pro End Bearing Mount (Bolt):1
- Mate:738: Hex Bearing 1-2 in (FR8ZZ-Hex, am-0279):10 ↔ Vex Pro End Bearing Mount (Bolt):1
- Mate:739: Hex Bearing 1-2 in (FR8ZZ-Hex, am-0279):10 ↔ Vex Pro End Bearing Mount (Bolt):1
- Mate:740: Bearing Mount Spacer 1-8 in:5 ↔ Vex Pro End Bearing Mount (Bolt):2
- Mate:741: Bearing Mount Spacer 1-8 in:5 ↔ Vex Pro End Bearing Mount (Bolt):2
- Mate:742: Bearing Mount Spacer 1-8 in:5 ↔ Vex Pro End Bearing Mount (Bolt):2
- Flush:23 (-9.525 mm): Hex Bearing 1-2 in (FR8ZZ-Hex, am-0279):7 ↔ Hex Shaft 1-2 in (am-0856):4
- Mate:743: Bearing Mount Spacer 1-8 in:3 ↔ Vex Pro End Bearing Mount (Bolt):3
- Mate:744: Bearing Mount Spacer 1-8 in:3 ↔ Vex Pro End Bearing Mount (Bolt):3
- Mate:745: Bearing Mount Spacer 1-8 in:3 ↔ Vex Pro End Bearing Mount (Bolt):3
- Mate:746: Hex Bearing 1-2 in (FR8ZZ-Hex, am-0279):8 ↔ Vex Pro End Bearing Mount (Bolt):3
- Mate:747: Hex Bearing 1-2 in (FR8ZZ-Hex, am-0279):8 ↔ Vex Pro End Bearing Mount (Bolt):3
- Mate:748: Bearing Mount Spacer 1-8 in:1 ↔ Vex Pro End Bearing Mount (Bolt):4
- Mate:749: Bearing Mount Spacer 1-8 in:1 ↔ Vex Pro End Bearing Mount (Bolt):4
- Mate:750: Bearing Mount Spacer 1-8 in:1 ↔ Vex Pro End Bearing Mount (Bolt):4
- Mate:752: Hex Bearing 1-2 in (FR8ZZ-Hex, am-0279):9 ↔ Vex Pro End Bearing Mount (Bolt):2
- Mate:753: Hex Bearing 1-2 in (FR8ZZ-Hex, am-0279):9 ↔ Vex Pro End Bearing Mount (Bolt):2
- Mate:754: Hex Bearing 1-2 in (FR8ZZ-Hex, am-0279):7 ↔ Vex Pro End Bearing Mount (Bolt):4
- Mate:755: Hex Bearing 1-2 in (FR8ZZ-Hex, am-0279):7 ↔ Vex Pro End Bearing Mount (Bolt):4
- Mate:758: Hex Bearing 1-2 in (FR8ZZ-Hex, am-0279):5 ↔ Hex Shaft Aluminum 1-2 in (am-2291):2
- Mate:759: Hex Bearing 1-2 in (FR8ZZ-Hex, am-0279):5 ↔ Hex Shaft Aluminum 1-2 in (am-2291):2
- Mate:774: Hex Shaft 1-2 in (am-0856):4 ↔ Hex Bearing 1-2 in (FR8ZZ-Hex, am-0279):8
- Mate:775: Hex Shaft 1-2 in (am-0856):5 ↔ Hex Bearing 1-2 in (FR8ZZ-Hex, am-0279):10
- Mate:790: Vex Pro 1x1 rectangular tubing 14 in length (roller):1 ↔ Bracket:1
- Mate:791: Vex Pro 1x1 rectangular tubing 14 in length (roller):1 ↔ Bracket:1
- Mate:793: Vex Pro 1x1 rectangular tubing 14 in length (roller):1 ↔ Bracket:1
- Mate:797: Hex Bearing 1-2 in (FR8ZZ-Hex, am-0279):3 ↔ Hex Shaft Aluminum 1-2 in (am-2291):1
- Mate:798: Vex Pro End Bearing Mount:4 ↔ Vex Pro 1x1 rectangular tubing 14 in length (roller):1
- Mate:799: Vex Pro End Bearing Mount:4 ↔ Vex Pro 1x1 rectangular tubing 14 in length (roller):1
- Mate:800: Vex Pro End Bearing Mount:5 ↔ Vex Pro 1x1 rectangular tubing 14 in length (roller):1
- Mate:801: Vex Pro End Bearing Mount:5 ↔ Vex Pro 1x1 rectangular tubing 14 in length (roller):1
- Mate:802: Vex Pro End Bearing Mount:8 ↔ Vex Pro 1x1 rectangular tubing 14 in length (roller):2
- Mate:803: Vex Pro End Bearing Mount:8 ↔ Vex Pro 1x1 rectangular tubing 14 in length (roller):2
- Mate:804: Vex Pro End Bearing Mount:7 ↔ Vex Pro 1x1 rectangular tubing 14 in length (roller):2
- Mate:805: Vex Pro End Bearing Mount:7 ↔ Vex Pro 1x1 rectangular tubing 14 in length (roller):2
- Mate:806: Vex Pro 1x1 rectangular tubing 14 in length (roller):2 ↔ Bracket:2
- Mate:807: Vex Pro 1x1 rectangular tubing 14 in length (roller):2 ↔ Bracket:2
- Mate:808: Vex Pro 1x1 rectangular tubing 14 in length (roller):2 ↔ Bracket:2
- Mate:809: Vex Pro 1x1 rectangular tubing 14 in length (roller):2 ↔ Bracket:3
- Mate:810: Vex Pro 1x1 rectangular tubing 14 in length (roller):2 ↔ Bracket:3
- Mate:811: Vex Pro 1x1 rectangular tubing 14 in length (roller):2 ↔ Bracket:3
- Flush:25: Vex Pro 1x1 rectangular tubing 2 in length:1 ↔ Vex Pro 1x1 rectangular tubing 2 in length:3
- Mate:829: Hex Shaft 1-2 in (am-0856):4 ↔ Hex Shaft Collar 1-2 in (7552K500):25
- Mate:830: Hex Bearing 1-2 in (FR8ZZ-Hex, am-0279):7 ↔ Hex Shaft Collar 1-2 in (7552K500):25
- Mate:831: Hex Shaft 1-2 in (am-0856):4 ↔ Hex Shaft Collar 1-2 in (7552K500):25
- Mate:832: Hex Bearing 1-2 in (FR8ZZ-Hex, am-0279):8 ↔ Hex Shaft Collar 1-2 in (7552K500):26
- Mate:833: Hex Shaft 1-2 in (am-0856):4 ↔ Hex Shaft Collar 1-2 in (7552K500):26
- Mate:834: Hex Shaft 1-2 in (am-0856):4 ↔ Hex Shaft Collar 1-2 in (7552K500):26
- Mate:835: Hex Bearing 1-2 in (FR8ZZ-Hex, am-0279):10 ↔ Hex Shaft Collar 1-2 in (7552K500):27
- Mate:836: Hex Shaft 1-2 in (am-0856):5 ↔ Hex Shaft Collar 1-2 in (7552K500):27
- Mate:843: Hex Shaft 1-2 in (am-0856):5 ↔ Hex Shaft Collar 1-2 in (7552K500):27
- Mate:852: Hex Shaft 1-2 in (am-0856):5 ↔ Hex Shaft Collar 1-2 in (7552K500):29
- Mate:853: Hex Shaft 1-2 in (am-0856):5 ↔ Hex Shaft Collar 1-2 in (7552K500):29
- Mate:854: Hex Bearing 1-2 in (FR8ZZ-Hex, am-0279):9 ↔ Hex Shaft Collar 1-2 in (7552K500):29
- Mate:856: Bracket:2 ↔ Shaft Collar 3-16 in ID (6435K510):2
- Mate:858: Bracket:3 ↔ Shaft Collar 3-16 in ID (6435K510):1
- Mate:860: Bracket:1 ↔ Shaft Collar 3-16 in ID (6435K510):3
- Mate:862: Vex Pro 1x1 rectangular tubing 14 in length (roller):1 ↔ Bracket:4
- Mate:863: Vex Pro 1x1 rectangular tubing 14 in length (roller):1 ↔ Bracket:4
- Mate:864: Vex Pro 1x1 rectangular tubing 14 in length (roller):1 ↔ Bracket:4
- Mate:865: Shaft Collar 3-16 in ID (6435K510):4 ↔ Bracket:4
- Mate:866: Vex Pro End Bearing Mount:5 ↔ Standoff #8 (91125A459):1
- Mate:867: Vex Pro End Bearing Mount:5 ↔ Standoff #8 (91125A459):1
- Mate:868: Vex Pro End Bearing Mount:5 ↔ Standoff #8 (91125A459):2
- Mate:869: Vex Pro End Bearing Mount:5 ↔ Standoff #8 (91125A459):2
- Mate:870: Vex Pro End Bearing Mount:5 ↔ Standoff #8 (91125A459):3
- Mate:871: Vex Pro End Bearing Mount:5 ↔ Standoff #8 (91125A459):3
- Mate:872: Vex Pro End Bearing Mount:5 ↔ Standoff #8 (91125A459):4
- Mate:873: Vex Pro End Bearing Mount:4 ↔ Standoff #8 (91125A459):4
- Mate:874: Vex Pro End Bearing Mount:8 ↔ Standoff #8 (91125A459):5
- Mate:875: Vex Pro End Bearing Mount:8 ↔ Standoff #8 (91125A459):5
- Mate:876: Vex Pro End Bearing Mount:8 ↔ Standoff #8 (91125A459):6
- Mate:877: Vex Pro End Bearing Mount:8 ↔ Standoff #8 (91125A459):6
- Mate:878: Vex Pro End Bearing Mount:8 ↔ Standoff #8 (91125A459):7
- Mate:879: Vex Pro End Bearing Mount:8 ↔ Standoff #8 (91125A459):7
- Mate:880: Vex Pro End Bearing Mount:8 ↔ Standoff #8 (91125A459):8
- Mate:881: Vex Pro End Bearing Mount:8 ↔ Standoff #8 (91125A459):8
- Mate:887: Vex Pro 1x1 rectangular tubing 14 in length (roller):1 ↔ Roller Crossbar Gusset (Custom):2
- Mate:892: Vex Pro 1x1 rectangular tubing 14 in length (roller):2 ↔ Roller Crossbar Gusset (Custom):4
- Mate:894: Vex Pro 1x1 rectangular tubing 21.375 in length:1 ↔ Roller Crossbar Gusset (Custom):4
- Mate:896: Vex Pro 1x1 rectangular tubing 14 in length (roller):2 ↔ Roller Crossbar Gusset (Custom):3
- Mate:897: Vex Pro 1x1 rectangular tubing 21.375 in length:1 ↔ Roller Crossbar Gusset (Custom):3
- Mate:900: Vex Pro 1x1 rectangular tubing 21.375 in length:1 ↔ Roller Crossbar Gusset (Custom):2
- Mate:901: Vex Pro 1x1 rectangular tubing 21.375 in length:1 ↔ Roller Crossbar Gusset (Custom):2
- Mate:902: Vex Pro 1x1 rectangular tubing 21.375 in length:1 ↔ Roller Crossbar Gusset (Custom):2
- Mate:903: Vex Pro 1x1 rectangular tubing 14 in length (roller):1 ↔ Roller Crossbar Gusset (Custom):2
- Mate:904: Vex Pro 1x1 rectangular tubing 14 in length (roller):1 ↔ Roller Crossbar Gusset (Custom):2
- Mate:905: Vex Pro 1x1 rectangular tubing 14 in length (roller):2 ↔ Roller Crossbar Gusset (Custom):3
- Mate:906: Vex Pro 1x1 rectangular tubing 14 in length (roller):2 ↔ Roller Crossbar Gusset (Custom):3
- Mate:907: Vex Pro 1x1 rectangular tubing 14 in length (roller):2 ↔ Roller Crossbar Gusset (Custom):4
- Mate:908: Vex Pro 1x1 rectangular tubing 14 in length (roller):2 ↔ Roller Crossbar Gusset (Custom):4
- Mate:909: Vex Pro 1x1 rectangular tubing 14 in length (roller):1 ↔ Roller Crossbar Gusset (Custom):5
- Mate:910: Vex Pro 1x1 rectangular tubing 14 in length (roller):1 ↔ Roller Crossbar Gusset (Custom):5
- Mate:911: Vex Pro 1x1 rectangular tubing 21.375 in length:1 ↔ Roller Crossbar Gusset (Custom):5
- Mate:912: Vex Pro 1x1 rectangular tubing 14 in length (roller):1 ↔ Roller Crossbar Gusset (Custom):5
- Mate:915: Hex Shaft 3-8 in (am-0855):2 ↔ Hex Shaft Collar 3-8 in (7552K300):5
- Mate:916: Clamp with Piston Assembly:2 ↔ Hex Shaft Collar 3-8 in (7552K300):5
- Mate:917: Hex Shaft 3-8 in (am-0855):2 ↔ Hex Shaft Collar 3-8 in (7552K300):5
- Mate:918: Clamp with Piston Assembly:1 ↔ Hex Shaft Collar 3-8 in (7552K300):6
- Mate:919: Hex Shaft 3-8 in (am-0855):1 ↔ Hex Shaft Collar 3-8 in (7552K300):6
- Mate:920: Hex Shaft 3-8 in (am-0855):1 ↔ Hex Shaft Collar 3-8 in (7552K300):6
- Mate:921: Clamp with Piston Assembly:1 ↔ Hex Shaft Collar 3-8 in (7552K300):7
- Mate:922: Hex Shaft 3-8 in (am-0855):1 ↔ Hex Shaft Collar 3-8 in (7552K300):7
- Mate:923: Hex Shaft 3-8 in (am-0855):1 ↔ Hex Shaft Collar 3-8 in (7552K300):7
- Mate:924: Clamp with Piston Assembly:2 ↔ Hex Shaft Collar 3-8 in (7552K300):8
- Mate:925: Hex Shaft 3-8 in (am-0855):2 ↔ Hex Shaft Collar 3-8 in (7552K300):8
- Mate:926: Hex Shaft 3-8 in (am-0855):2 ↔ Hex Shaft Collar 3-8 in (7552K300):8
- Mate:929: Pneumatic Piston Front Flange (Lt Custom):1 ↔ Vex Pro 1x1 rectangular tubing 2 in length (Flange Support):1
- Mate:930: Pneumatic Piston Front Flange (Lt Custom):1 ↔ Vex Pro 1x1 rectangular tubing 2 in length (Flange Support):1
- Mate:931: Pneumatic Piston Front Flange (Lt Custom):1 ↔ Vex Pro 1x1 rectangular tubing 2 in length (Flange Support):1
- Mate:932: Pneumatic Piston Front Flange (Rt Custom):2 ↔ Vex Pro 1x1 rectangular tubing 2 in length (Flange Support):2
- Mate:933: Pneumatic Piston Front Flange (Rt Custom):2 ↔ Vex Pro 1x1 rectangular tubing 2 in length (Flange Support):2
- Mate:934: Pneumatic Piston Front Flange (Rt Custom):2 ↔ Vex Pro 1x1 rectangular tubing 2 in length (Flange Support):2
- Mate:935: Vex Pro 1x1 rectangular tubing 14 in length:6 ↔ Vex Pro 90 degree gusset (1-8 in):1
- Mate:936: Vex Pro 1x1 rectangular tubing 14 in length:6 ↔ Vex Pro 90 degree gusset (1-8 in):1
- Mate:937: Vex Pro 1x1 rectangular tubing 2 in length:3 ↔ Vex Pro 90 degree gusset (1-8 in):1
- Mate:938: Vex Pro 1x1 rectangular tubing 14 in length:6 ↔ Vex Pro 90 degree gusset (1-8 in):1
- Mate:939: Vex Pro 90 degree gusset:15 ↔ Vex Pro 90 degree gusset (1-8 in):2
- Mate:940: Vex Pro 1x1 rectangular tubing 14 in length:5 ↔ Vex Pro 90 degree gusset (1-8 in):2
- Mate:941: Vex Pro 1x1 rectangular tubing 2 in length:1 ↔ Vex Pro 90 degree gusset (1-8 in):2
- Mate:942: Vex Pro 1x1 rectangular tubing 14 in length:5 ↔ Vex Pro 90 degree gusset (1-8 in):2
- Mate:945: Hex Shaft Collar 1-2 in (7552K500):20 ↔ Timing Pulley (HTD 5mm) - 18T 15mm 1-2 in Hex:1
- Mate:946: Hex Shaft 1-2 in 5 in long (am-0856):1 ↔ Timing Pulley (HTD 5mm) - 18T 15mm 1-2 in Hex:1
- Mate:947: Hex Shaft 1-2 in 5 in long (am-0856):1 ↔ Timing Pulley (HTD 5mm) - 18T 15mm 1-2 in Hex:1
- Mate:948: Hex Shaft Collar 1-2 in (7552K500):24 ↔ Timing Pulley (HTD 5mm) - 18T 15mm 1-2 in Hex:1
- Mate:949: Vex Pro 1x1 rectangular tubing 2 in length:3 ↔ Hex Spacer:1
- Mate:950: Vex Pro 1x1 rectangular tubing 2 in length:3 ↔ Hex Spacer:1
- Mate:951: Hex Shaft 3-8 in (am-0855):2 ↔ Hex Spacer:1
- Mate:952: Vex Pro 1x1 rectangular tubing 2 in length:3 ↔ Hex Spacer:2
- Mate:953: Vex Pro 1x1 rectangular tubing 2 in length:3 ↔ Hex Spacer:2
- Mate:954: Hex Shaft 3-8 in (am-0855):2 ↔ Hex Spacer:2
- Mate:955: Vex Pro 1x1 rectangular tubing 2 in length:4 ↔ Hex Spacer:3
- Mate:956: Vex Pro 1x1 rectangular tubing 2 in length:4 ↔ Hex Spacer:3
- Mate:957: Hex Shaft 3-8 in (am-0855):2 ↔ Hex Spacer:3
- Mate:958: Vex Pro 1x1 rectangular tubing 2 in length:4 ↔ Hex Spacer:4
- Mate:959: Vex Pro 1x1 rectangular tubing 2 in length:4 ↔ Hex Spacer:4
- Mate:960: Hex Shaft 3-8 in (am-0855):2 ↔ Hex Spacer:4
- Mate:961: Vex Pro 1x1 rectangular tubing 2 in length:1 ↔ Hex Spacer:5
- Mate:962: Vex Pro 1x1 rectangular tubing 2 in length:1 ↔ Hex Spacer:5
- Mate:963: Hex Shaft 3-8 in (am-0855):1 ↔ Hex Spacer:5
- Mate:964: Vex Pro 1x1 rectangular tubing 2 in length:1 ↔ Hex Spacer:6
- Mate:965: Vex Pro 1x1 rectangular tubing 2 in length:1 ↔ Hex Spacer:6
- Mate:966: Hex Shaft 3-8 in (am-0855):1 ↔ Hex Spacer:6
- Mate:967: Vex Pro 1x1 rectangular tubing 2 in length:2 ↔ Hex Spacer:7
- Mate:968: Vex Pro 1x1 rectangular tubing 2 in length:2 ↔ Hex Spacer:7
- Mate:969: Hex Shaft 3-8 in (am-0855):1 ↔ Hex Spacer:7
- Mate:970: Vex Pro 1x1 rectangular tubing 2 in length:2 ↔ Hex Spacer:8
- Mate:971: Vex Pro 1x1 rectangular tubing 2 in length:2 ↔ Hex Spacer:8
- Mate:972: Hex Shaft 3-8 in (am-0855):1 ↔ Hex Spacer:8
- Mate:973: Vex Pro 1x1 rectangular tubing 14 in length:6 ↔ Bearing Mount Spacer 1-8 in:1
- Mate:974: Vex Pro 1x1 rectangular tubing 14 in length:6 ↔ Bearing Mount Spacer 1-8 in:3
- Mate:975: Vex Pro 1x1 rectangular tubing 14 in length:5 ↔ Bearing Mount Spacer 1-8 in:7
- Mate:976: Vex Pro 1x1 rectangular tubing 14 in length:6 ↔ Bearing Mount Spacer 1-8 in:1
- Mate:977: Vex Pro 1x1 rectangular tubing 14 in length:6 ↔ Vex Pro End Bearing Mount (Bolt):4
- Mate:978: Vex Pro 1x1 rectangular tubing 14 in length:6 ↔ Bearing Mount Spacer 1-8 in:3
- Mate:979: Vex Pro 1x1 rectangular tubing 14 in length:5 ↔ Vex Pro End Bearing Mount (Bolt):1
- Mate:980: Bearing Mount Spacer 1-8 in:7 ↔ Vex Pro End Bearing Mount (Bolt):1
- Mate:981: Vex Pro 1x1 rectangular tubing 14 in length:5 ↔ Vex Pro End Bearing Mount (Bolt):2
- Mate:983: Vex Pro 1x1 rectangular tubing 14 in length:5 ↔ Bearing Mount Spacer 1-8 in:5
- Mate:988: Vex Pro 1x1 rectangular tubing 14 in length (roller):1 ↔ Side Mount Custom:1
- Mate:989: Vex Pro 1x1 rectangular tubing 14 in length (roller):1 ↔ Side Mount Custom:1
- Mate:990: VersaPlanetary (Fixed):1 ↔ Side Mount Custom:1
- Mate:991: VersaPlanetary (Fixed):1 ↔ Side Mount Custom:1
- Mate:992: VersaPlanetary (Fixed):1 ↔ Side Mount Custom:1
- Mate:1020: Vex Pro 1x1 rectangular tubing 14 in length:6 ↔ Vex Pro 90 degree gusset:18
- Mate:1021: Vex Pro 1x1 rectangular tubing 14 in length:6 ↔ Vex Pro 90 degree gusset:18
- Mate:1022: Vex Pro 1x1 rectangular tubing 14 in length:5 ↔ Vex Pro 90 degree gusset:15
- Mate:1023: Vex Pro 1x1 rectangular tubing 14 in length:5 ↔ Vex Pro 90 degree gusset:15
- Mate:1024: Pneumatic Piston Back Flange (Right Custom):1 ↔ Clamp Piston ( 1 in stroke twice, 9-16 bore):1
- Mate:1025: Pneumatic Piston Back Flange (Right Custom):1 ↔ Clamp Piston ( 1 in stroke twice, 9-16 bore):1
- Mate:1026: Pneumatic Piston Back Flange (Right Custom):1 ↔ Clamp Piston ( 1 in stroke twice, 9-16 bore):1
- Mate:1028: Pneumatic Piston Back Flange (Rt Custom):1 ↔ Clamp Piston ( 1 in stroke twice, 9-16 bore):2
- Mate:1029: Pneumatic Piston Back Flange (Rt Custom):1 ↔ Clamp Piston ( 1 in stroke twice, 9-16 bore):2
- Mate:1030: Pneumatic Piston Back Flange (Rt Custom):1 ↔ Clamp Piston ( 1 in stroke twice, 9-16 bore):2
- Mate:1032: Hex Shaft 1-2 in 5 in long (am-0856):1 ↔ Hex Shaft Collar 1-2 in (7552K500):30
- Mate:1033: Hex Shaft 1-2 in 5 in long (am-0856):1 ↔ Hex Shaft Collar 1-2 in (7552K500):30
- Mate:1034: Gusset 3 (R-L) (Custom):1 ↔ Hex Shaft Collar 1-2 in (7552K500):30
- Mate:1036: Vex Pro 1x1 rectangular tubing 14 in length (roller):2 ↔ Hex Spacer:9
- Mate:1037: Hex Shaft 1-2 in (am-0856):5 ↔ Hex Spacer:9